# Autodesk Inventor assembly: subflap
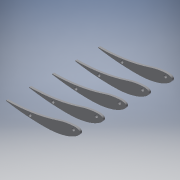
[picture p0: Inventor's stored thumbnail of the model, 180x180]
Saved by Autodesk Inventor 2018.2 (Build 222227000, 227)
## iProperties
Created: 2018-03-14
Part Number: subflap
Material: 一般
Document SubType Name: Assembly
Designer: ku_sk
Author: ku_sk
## Documents named in this file (2)
- C:\Users\ku_sk\Documents\Inventor\Aero\KS-15\Rr.wing\parts\subflap\subflap.iam
- C:\Users\ku_sk\Documents\Inventor\Aero\KS-15\Rr.wing\parts\flap_s.ipt
## Components (5 placed, 1 different names)
1. flap_s:1 — メイト:2, メイト:11, メイト:12
2. flap_s:2 — メイト:1, メイト:2, メイト:9, メイト:10, メイト:11, メイト:12
3. flap_s:3 — メイト:1, メイト:3, メイト:5, メイト:6, メイト:9, メイト:10, フラッシュ:1, 角度:1, メイト:13
4. flap_s:4 — メイト:3, メイト:4, メイト:5, メイト:6, メイト:7, メイト:8
5. flap_s:5 — メイト:4, メイト:7, メイト:8
## Relationships (15: Mate 13, Flush 1, Angle 1)
- メイト:1 [Mate] (41.5 mm): flap_s:2 ↔ flap_s:3
- メイト:2 [Mate] (41.5 mm): flap_s:1 ↔ flap_s:2
- メイト:3 [Mate] (41.5 mm): flap_s:3 ↔ flap_s:4
- メイト:4 [Mate] (41.5 mm): flap_s:4 ↔ flap_s:5
- メイト:5 [Mate]: flap_s:3 ↔ flap_s:4
- メイト:6 [Mate]: flap_s:3 ↔ flap_s:4
- メイト:7 [Mate]: flap_s:4 ↔ flap_s:5
- メイト:8 [Mate]: flap_s:4 ↔ flap_s:5
- メイト:9 [Mate]: flap_s:2 ↔ flap_s:3
- メイト:10 [Mate]: flap_s:2 ↔ flap_s:3
- メイト:11 [Mate]: flap_s:1 ↔ flap_s:2
- メイト:12 [Mate]: flap_s:1 ↔ flap_s:2
- フラッシュ:1 [Flush]: flap_s:3
- 角度:1 [Angle] (0 deg): flap_s:3
- メイト:13 [Mate]: flap_s:3
